# Autodesk Inventor assembly: !conveyer_box
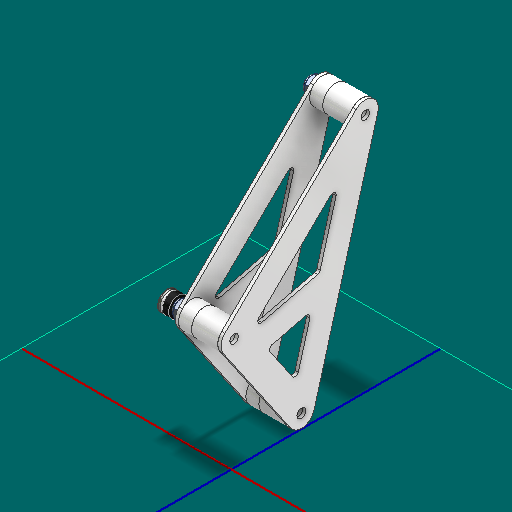
[picture p0: Inventor's stored thumbnail of the model, 512x512]
Saved by Autodesk Inventor 2025 (Build 290162000, 162)
## iProperties
Created: 2024-08-19
Part Number: !conveyer_box
Document SubType Name: Assembly
Designer: averey
Author: averey
## Documents named in this file (14)
- C:\Users\avere\vex_robotics_high_stakes\hardware\cad\ATLAS\tower\conveyer_box\structure.iam
- structure.iam
- C:\Users\avere\vex_robotics_high_stakes\hardware\cad\ATLAS\tower\conveyer_box\custom_parts\gusset.ipt
- C:\Users\avere\vex_robotics_high_stakes\hardware\cad\VEX-CAD-Inventor\Motion\Spacers\Spacer Nylon .500 OD\NSpacer White .500 OD x .250.ipt
- C:\Users\avere\vex_robotics_high_stakes\hardware\cad\VEX-CAD-Inventor\Motion\Spacers\Spacer Nylon .500 OD.ipt
- C:\Users\avere\vex_robotics_high_stakes\hardware\cad\VEX-CAD-Inventor\Motion\Spacers\Spacer Nylon .500 OD\NSpacer White .500 OD x .500.ipt
- C:\Users\avere\vex_robotics_high_stakes\hardware\cad\VEX-CAD-Inventor\Structure\Hardware\Nut Thin Nylock.ipt
- C:\Users\avere\vex_robotics_high_stakes\hardware\cad\VEX-CAD-Inventor\Motion\Spacers\Spacer Nylon .375 OD\NSpacer .375 OD x .125.ipt
- C:\Users\avere\vex_robotics_high_stakes\hardware\cad\VEX-CAD-Inventor\Motion\Spacers\Spacer Nylon .375 OD.ipt
- C:\Users\avere\vex_robotics_high_stakes\hardware\cad\VEX-CAD-Inventor\Motion\Spacers\Washer Steel\SWasher .375 OD x .015625.ipt
- C:\Users\avere\vex_robotics_high_stakes\hardware\cad\VEX-CAD-Inventor\Motion\Spacers\Washer Steel.ipt
- C:\Users\avere\vex_robotics_high_stakes\hardware\cad\VEX-CAD-Inventor\Motion\Spacers\Washer Steel\SWasher .375 OD x .031250.ipt
- C:\Users\avere\vex_robotics_high_stakes\hardware\cad\VEX-CAD-Inventor\Motion\Spacers\Washer Teflon\TWasher .375 OD x .04000.ipt
- C:\Users\avere\vex_robotics_high_stakes\hardware\cad\VEX-CAD-Inventor\Motion\Spacers\Washer Teflon.ipt
## Components (14 placed, 8 different names)
1. gusset:1 — Insert:1, Insert:8, Insert:9
2. gusset:2 — Mate:2, Insert:1, Insert:5, Insert:6, Insert:7
3. NSpacer White .500 OD x .250:1 — Insert:4
4. NSpacer White .500 OD x .500:2 — Insert:4, Insert:6
5. NSpacer White .500 OD x .250:3 — Insert:3
6. NSpacer White .500 OD x .500:4 — Insert:3, Insert:7
7. NSpacer White .500 OD x .250:5 — Insert:2
8. NSpacer White .500 OD x .500:6 — Insert:2, Insert:5
9. Nut Thin Nylock:1 — Insert:8, Insert:13
10. Nut Thin Nylock:2 — Insert:9
11. NSpacer .375 OD x .125:1 — Insert:12, Insert:13
12. SWasher .375 OD x .015625:1 — Insert:10
13. SWasher .375 OD x .031250:2 — Insert:10, Insert:11
14. TWasher .375 OD x .04000:1 — Insert:11, Insert:12
## Relationships (15: Insert 13, Mate 2)
- [Mate]: gusset:1 ↔ gusset:2
- Mate:2: gusset:2
- Insert:1 (19.05 mm): gusset:1 ↔ gusset:2
- Insert:2: NSpacer White .500 OD x .250:5 ↔ NSpacer White .500 OD x .500:6
- Insert:3: NSpacer White .500 OD x .250:3 ↔ NSpacer White .500 OD x .500:4
- Insert:4: NSpacer White .500 OD x .250:1 ↔ NSpacer White .500 OD x .500:2
- Insert:5: gusset:2 ↔ NSpacer White .500 OD x .500:6
- Insert:6: gusset:2 ↔ NSpacer White .500 OD x .500:2
- Insert:7: gusset:2 ↔ NSpacer White .500 OD x .500:4
- Insert:8: gusset:1 ↔ Nut Thin Nylock:1
- Insert:9: gusset:1 ↔ Nut Thin Nylock:2
- Insert:10: SWasher .375 OD x .015625:1 ↔ SWasher .375 OD x .031250:2
- Insert:11: SWasher .375 OD x .031250:2 ↔ TWasher .375 OD x .04000:1
- Insert:12: NSpacer .375 OD x .125:1 ↔ TWasher .375 OD x .04000:1
- Insert:13: Nut Thin Nylock:1 ↔ NSpacer .375 OD x .125:1
